# Autodesk Inventor assembly: SCARA
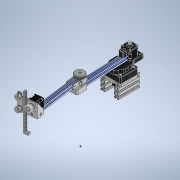
[picture p0: Inventor's stored thumbnail of the model, 180x180]
Saved by Autodesk Inventor 2022 (Build 260153000, 153)
## iProperties
Created: 2022-03-02
Part Number: SCARA
Document SubType Name: Assembly
Designer: JK
Author: JK
## Documents named in this file (4)
- C:\Users\JK\Documents\Inventor\ScaraNema\SCARA-3DP\Parts\SCARA.iam
- C:\Users\JK\Documents\Inventor\ScaraNema\SCARA-3DP\Parts\Shoulder\Shoulder base.iam
- C:\Users\JK\Documents\Inventor\ScaraNema\SCARA-3DP\Parts\Elbow\Elbow assembly.iam
- C:\Users\JK\Documents\Inventor\ScaraNema\SCARA-3DP\Parts\Z axis\Z assembly.iam
## Components (3 placed, 3 different names)
1. Shoulder base:1 [sub-assembly] — Coincidencia:1, Coincidencia:2
2. Elbow assembly:1 [sub-assembly] — Coincidencia:1, Coincidencia:2, Coincidencia:3, Coincidencia:4, Coincidencia:5
3. Z assembly:1 [sub-assembly] — Coincidencia:3, Coincidencia:4, Coincidencia:5
## Relationships (5: Mate 5)
- Coincidencia:1 [Mate]: Shoulder base:1 ↔ Elbow assembly:1
- Coincidencia:2 [Mate]: Shoulder base:1 ↔ Elbow assembly:1
- Coincidencia:3 [Mate]: Elbow assembly:1 ↔ Z assembly:1
- Coincidencia:4 [Mate] (0.15 mm): Elbow assembly:1 ↔ Z assembly:1
- Coincidencia:5 [Mate]: Elbow assembly:1 ↔ Z assembly:1
